# Autodesk Inventor assembly: Placa_Juguete
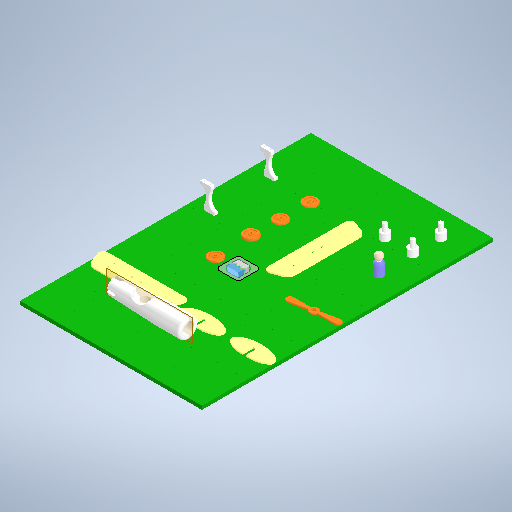
[picture p0: Inventor's stored thumbnail of the model, 512x512]
Saved by Autodesk Inventor 2025.2 (Build 292293000, 293)
## iProperties
Created: 2025-03-01
Part Number: Placa_Juguete
Document SubType Name: Assembly
Designer: hmont
Author: hmont
## Documents named in this file (10)
- C:\Users\hmont\OneDrive\Desktop\2024-2\Automatizacion de Procesos de Manufactura\Juguete\Placa_Juguete.iam
- C:\Users\hmont\OneDrive\Desktop\2024-2\Automatizacion de Procesos de Manufactura\Juguete\Placa.ipt
- C:\Users\hmont\Downloads\wooden-toy-plane-biplane-pdf-1.snapshot.3\LowerWing\LowerWing\LowerWing.ipt
- C:\Users\hmont\Downloads\wooden-toy-plane-biplane-pdf-1.snapshot.3\HorizontalTail\HorizontalTail\HorizontalTail.ipt
- C:\Users\hmont\Downloads\wooden-toy-plane-biplane-pdf-1.snapshot.3\Pilot\Pilot\Pilot.ipt
- C:\Users\hmont\Downloads\wooden-toy-plane-biplane-pdf-1.snapshot.3\Wheel\Wheel\Wheel.ipt
- C:\Users\hmont\Downloads\wooden-toy-plane-biplane-pdf-1.snapshot.3\Propellor\Propellor\Propellor.ipt
- C:\Users\hmont\Downloads\wooden-toy-plane-biplane-pdf-1.snapshot.3\Motor\Motor\Motor.ipt
- C:\Users\hmont\Downloads\wooden-toy-plane-biplane-pdf-1.snapshot.3\VerticalCrossbar\VerticalCrossbar\VerticalCrossbar.ipt
- C:\Users\hmont\Downloads\wooden-toy-plane-biplane-pdf-1.snapshot.3\Fuselage\Fuselage\Fuselage.ipt
## Components (17 placed, 9 different names)
1. Placa:1 — Rígido:1, Rígido:2, Rígido:3, Rígido:4, Rígido:5, Rígido:6, Rígido:7, Rígido:8, Rígido:9, Rígido:10, Rígido:11, Rígido:12, Rígido:13, Rígido:14, Rígido:15, Rígido:16
2. LowerWing:1 — Rígido:1
3. LowerWing:2 — Rígido:6
4. HorizontalTail:1 — Rígido:7
5. HorizontalTail:2 — Rígido:8
6. Pilot:1 — Rígido:10
7. Wheel:1 — Rígido:4
8. Wheel:2 — Rígido:3
9. Wheel:3 — Rígido:2
10. Wheel:4 — Rígido:5
11. Propellor:1 — Rígido:9
12. Motor:1 — Rígido:13
13. Motor:2 — Rígido:12
14. Motor:3 — Rígido:11
15. VerticalCrossbar:1 — Rígido:15
16. VerticalCrossbar:2 — Rígido:14
17. Fuselage:1 — Rígido:16
## Relationships (16: WeldJoint 16)
- Rígido:1 [WeldJoint] (3 mm): Placa:1 ↔ LowerWing:1
- Rígido:2 [WeldJoint] (3 mm): Placa:1 ↔ Wheel:3
- Rígido:3 [WeldJoint] (3 mm): Placa:1 ↔ Wheel:2
- Rígido:4 [WeldJoint] (3 mm): Placa:1 ↔ Wheel:1
- Rígido:5 [WeldJoint] (3 mm): Placa:1 ↔ Wheel:4
- Rígido:6 [WeldJoint] (3 mm): Placa:1 ↔ LowerWing:2
- Rígido:7 [WeldJoint] (3 mm): Placa:1 ↔ HorizontalTail:1
- Rígido:8 [WeldJoint] (3 mm): Placa:1 ↔ HorizontalTail:2
- Rígido:9 [WeldJoint] (3 mm): Placa:1 ↔ Propellor:1
- Rígido:10 [WeldJoint] (3 mm): Placa:1 ↔ Pilot:1
- Rígido:11 [WeldJoint] (3 mm): Placa:1 ↔ Motor:3
- Rígido:12 [WeldJoint] (3 mm): Placa:1 ↔ Motor:2
- Rígido:13 [WeldJoint] (3 mm): Placa:1 ↔ Motor:1
- Rígido:14 [WeldJoint] (3 mm): Placa:1 ↔ VerticalCrossbar:2
- Rígido:15 [WeldJoint] (3 mm): Placa:1 ↔ VerticalCrossbar:1
- Rígido:16 [WeldJoint] (20 mm): Placa:1 ↔ Fuselage:1
